# Autodesk Inventor assembly: 200-40-BOGIE-CONNECTOR-REINFORCEMENT-01
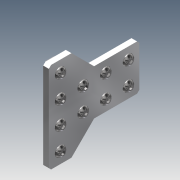
[picture p0: Inventor's stored thumbnail of the model, 180x180]
Saved by Autodesk Inventor 2018.2 (Build 222227000, 227)
## iProperties
Manager: feesmrt
Company: FRANCOR
Part Number: 200-40-BOGIE-CONNECTOR-REINFORCEMENT-01
Project: Rescue Robot
Cost Center: -
Material: Generisch
Document SubType Name: Assembly
Designer: feesmrt
Engineer: feesmrt
Authority: feesmrt
Description: Bogie Connector Verstärkung
Stock Number: 200-40-BOGIE-CONNECTOR-REINFORCEMENT-01
Subject: Rescue Robot
Author: feesmrt
Revision Number: 1
Title: Bogie Connector Verstärkung
## Documents named in this file (4)
- D:\Programmierung\FRANC0R\CAD\02-Rocker-Bogie-Robot\200-ROCKER-BOGIE\200-40-BOGIE-CONNECTOR\200-40-BOGIE-CONNECTOR-REINFORCEMENT-01.iam
- D:\Programmierung\FRANC0R\CAD\02-Rocker-Bogie-Robot\200-ROCKER-BOGIE\200-40-BOGIE-CONNECTOR\200-40-BOGIE-CONNECTOR-06.ipt
- D:\Programmierung\FRANC0R\CAD\02-Rocker-Bogie-Robot\900-COMPONENTS\900-50-PROFILES\900-50-PROFILES-CONN-N6xM5.ipt
- D:\Programmierung\FRANC0R\CAD\02-Rocker-Bogie-Robot\900-COMPONENTS\900-40-SCREWS\900-40-SCREWS-ISO7830_M5x10.ipt
## Components (21 placed, 3 different names)
1. 200-40-BOGIE-CONNECTOR-06:1 — Passend:1, Passend:2, Passend:3, Passend:4, Passend:5, Passend:6, Passend:7, Passend:8, Passend:9, Passend:10, Passend:11, Passend:12, Passend:13, Passend:14, Passend:15, Passend:16, Winkel:1, Winkel:2, Winkel:3, Winkel:4, Winkel:5, Winkel:6, Winkel:7, Winkel:8, Passend:25, Passend:26, Passend:27, Passend:28, Passend:29, Passend:30, Passend:31, Passend:32, Passend:33, Passend:34, Passend:35, Passend:36, Winkel:9, Winkel:10, Passend:39, Passend:40
2. 900-50-PROFILES-CONN-N6xM5:1 — Passend:1, Passend:9, Winkel:4, Passend:24
3. 900-50-PROFILES-CONN-N6xM5:2 — Passend:2, Passend:10, Winkel:3, Passend:23
4. 900-50-PROFILES-CONN-N6xM5:3 — Passend:3, Passend:11, Winkel:2, Passend:22
5. 900-50-PROFILES-CONN-N6xM5:4 — Passend:4, Passend:12, Winkel:1, Passend:21
6. 900-50-PROFILES-CONN-N6xM5:5 — Passend:5, Passend:13, Winkel:5, Passend:19
7. 900-50-PROFILES-CONN-N6xM5:6 — Passend:6, Passend:14, Winkel:7, Passend:20
8. 900-50-PROFILES-CONN-N6xM5:7 — Passend:7, Passend:16, Winkel:6, Passend:18
9. 900-50-PROFILES-CONN-N6xM5:8 — Passend:8, Passend:15, Winkel:8, Passend:17
10. 900-40-SCREWS-ISO7830_M5x10:1 — Passend:17, Passend:25
11. 900-40-SCREWS-ISO7830_M5x10:2 — Passend:18, Passend:26
12. 900-40-SCREWS-ISO7830_M5x10:3 — Passend:20, Passend:27
13. 900-40-SCREWS-ISO7830_M5x10:4 — Passend:19, Passend:28
14. 900-40-SCREWS-ISO7830_M5x10:5 — Passend:21, Passend:29
15. 900-40-SCREWS-ISO7830_M5x10:6 — Passend:22, Passend:30
16. 900-40-SCREWS-ISO7830_M5x10:7 — Passend:23, Passend:31
17. 900-40-SCREWS-ISO7830_M5x10:8 — Passend:24, Passend:32
18. 900-50-PROFILES-CONN-N6xM5:9 — Passend:33, Passend:35, Winkel:10, Passend:37
19. 900-50-PROFILES-CONN-N6xM5:10 — Passend:34, Passend:36, Winkel:9, Passend:38
20. 900-40-SCREWS-ISO7830_M5x10:9 — Passend:37, Passend:39
21. 900-40-SCREWS-ISO7830_M5x10:10 — Passend:38, Passend:40
## Relationships (50: Mate 40, Angle 10)
- Passend:1 [Mate]: 200-40-BOGIE-CONNECTOR-06:1 ↔ 900-50-PROFILES-CONN-N6xM5:1
- Passend:2 [Mate]: 200-40-BOGIE-CONNECTOR-06:1 ↔ 900-50-PROFILES-CONN-N6xM5:2
- Passend:3 [Mate]: 200-40-BOGIE-CONNECTOR-06:1 ↔ 900-50-PROFILES-CONN-N6xM5:3
- Passend:4 [Mate]: 200-40-BOGIE-CONNECTOR-06:1 ↔ 900-50-PROFILES-CONN-N6xM5:4
- Passend:5 [Mate]: 200-40-BOGIE-CONNECTOR-06:1 ↔ 900-50-PROFILES-CONN-N6xM5:5
- Passend:6 [Mate]: 200-40-BOGIE-CONNECTOR-06:1 ↔ 900-50-PROFILES-CONN-N6xM5:6
- Passend:7 [Mate]: 200-40-BOGIE-CONNECTOR-06:1 ↔ 900-50-PROFILES-CONN-N6xM5:7
- Passend:8 [Mate]: 200-40-BOGIE-CONNECTOR-06:1 ↔ 900-50-PROFILES-CONN-N6xM5:8
- Passend:9 [Mate] (1.5 mm): 200-40-BOGIE-CONNECTOR-06:1 ↔ 900-50-PROFILES-CONN-N6xM5:1
- Passend:10 [Mate] (1.5 mm): 200-40-BOGIE-CONNECTOR-06:1 ↔ 900-50-PROFILES-CONN-N6xM5:2
- Passend:11 [Mate] (1.5 mm): 200-40-BOGIE-CONNECTOR-06:1 ↔ 900-50-PROFILES-CONN-N6xM5:3
- Passend:12 [Mate] (1.5 mm): 200-40-BOGIE-CONNECTOR-06:1 ↔ 900-50-PROFILES-CONN-N6xM5:4
- Passend:13 [Mate] (1.5 mm): 200-40-BOGIE-CONNECTOR-06:1 ↔ 900-50-PROFILES-CONN-N6xM5:5
- Passend:14 [Mate] (1.5 mm): 200-40-BOGIE-CONNECTOR-06:1 ↔ 900-50-PROFILES-CONN-N6xM5:6
- Passend:15 [Mate] (1.5 mm): 200-40-BOGIE-CONNECTOR-06:1 ↔ 900-50-PROFILES-CONN-N6xM5:8
- Passend:16 [Mate] (1.5 mm): 200-40-BOGIE-CONNECTOR-06:1 ↔ 900-50-PROFILES-CONN-N6xM5:7
- Winkel:1 [Angle] (0 deg): 200-40-BOGIE-CONNECTOR-06:1 ↔ 900-50-PROFILES-CONN-N6xM5:4
- Winkel:2 [Angle] (0 deg): 200-40-BOGIE-CONNECTOR-06:1 ↔ 900-50-PROFILES-CONN-N6xM5:3
- Winkel:3 [Angle] (0 deg): 200-40-BOGIE-CONNECTOR-06:1 ↔ 900-50-PROFILES-CONN-N6xM5:2
- Winkel:4 [Angle] (0 deg): 200-40-BOGIE-CONNECTOR-06:1 ↔ 900-50-PROFILES-CONN-N6xM5:1
- Winkel:5 [Angle] (0 deg): 200-40-BOGIE-CONNECTOR-06:1 ↔ 900-50-PROFILES-CONN-N6xM5:5
- Winkel:6 [Angle] (0 deg): 200-40-BOGIE-CONNECTOR-06:1 ↔ 900-50-PROFILES-CONN-N6xM5:7
- Winkel:7 [Angle] (0 deg): 200-40-BOGIE-CONNECTOR-06:1 ↔ 900-50-PROFILES-CONN-N6xM5:6
- Winkel:8 [Angle] (0 deg): 200-40-BOGIE-CONNECTOR-06:1 ↔ 900-50-PROFILES-CONN-N6xM5:8
- Passend:17 [Mate]: 900-50-PROFILES-CONN-N6xM5:8 ↔ 900-40-SCREWS-ISO7830_M5x10:1
- Passend:18 [Mate]: 900-50-PROFILES-CONN-N6xM5:7 ↔ 900-40-SCREWS-ISO7830_M5x10:2
- Passend:19 [Mate]: 900-50-PROFILES-CONN-N6xM5:5 ↔ 900-40-SCREWS-ISO7830_M5x10:4
- Passend:20 [Mate]: 900-50-PROFILES-CONN-N6xM5:6 ↔ 900-40-SCREWS-ISO7830_M5x10:3
- Passend:21 [Mate]: 900-50-PROFILES-CONN-N6xM5:4 ↔ 900-40-SCREWS-ISO7830_M5x10:5
- Passend:22 [Mate]: 900-50-PROFILES-CONN-N6xM5:3 ↔ 900-40-SCREWS-ISO7830_M5x10:6
- Passend:23 [Mate]: 900-50-PROFILES-CONN-N6xM5:2 ↔ 900-40-SCREWS-ISO7830_M5x10:7
- Passend:24 [Mate]: 900-50-PROFILES-CONN-N6xM5:1 ↔ 900-40-SCREWS-ISO7830_M5x10:8
- Passend:25 [Mate]: 200-40-BOGIE-CONNECTOR-06:1 ↔ 900-40-SCREWS-ISO7830_M5x10:1
- Passend:26 [Mate]: 200-40-BOGIE-CONNECTOR-06:1 ↔ 900-40-SCREWS-ISO7830_M5x10:2
- Passend:27 [Mate]: 200-40-BOGIE-CONNECTOR-06:1 ↔ 900-40-SCREWS-ISO7830_M5x10:3
- Passend:28 [Mate]: 200-40-BOGIE-CONNECTOR-06:1 ↔ 900-40-SCREWS-ISO7830_M5x10:4
- Passend:29 [Mate]: 200-40-BOGIE-CONNECTOR-06:1 ↔ 900-40-SCREWS-ISO7830_M5x10:5
- Passend:30 [Mate]: 200-40-BOGIE-CONNECTOR-06:1 ↔ 900-40-SCREWS-ISO7830_M5x10:6
- Passend:31 [Mate]: 200-40-BOGIE-CONNECTOR-06:1 ↔ 900-40-SCREWS-ISO7830_M5x10:7
- Passend:32 [Mate]: 200-40-BOGIE-CONNECTOR-06:1 ↔ 900-40-SCREWS-ISO7830_M5x10:8
- Passend:33 [Mate]: 200-40-BOGIE-CONNECTOR-06:1 ↔ 900-50-PROFILES-CONN-N6xM5:9
- Passend:34 [Mate]: 200-40-BOGIE-CONNECTOR-06:1 ↔ 900-50-PROFILES-CONN-N6xM5:10
- Passend:35 [Mate] (1.5 mm): 200-40-BOGIE-CONNECTOR-06:1 ↔ 900-50-PROFILES-CONN-N6xM5:9
- Passend:36 [Mate] (1.5 mm): 200-40-BOGIE-CONNECTOR-06:1 ↔ 900-50-PROFILES-CONN-N6xM5:10
- Winkel:9 [Angle] (0 deg): 200-40-BOGIE-CONNECTOR-06:1 ↔ 900-50-PROFILES-CONN-N6xM5:10
- Winkel:10 [Angle] (0 deg): 200-40-BOGIE-CONNECTOR-06:1 ↔ 900-50-PROFILES-CONN-N6xM5:9
- Passend:37 [Mate]: 900-50-PROFILES-CONN-N6xM5:9 ↔ 900-40-SCREWS-ISO7830_M5x10:9
- Passend:38 [Mate]: 900-50-PROFILES-CONN-N6xM5:10 ↔ 900-40-SCREWS-ISO7830_M5x10:10
- Passend:39 [Mate]: 200-40-BOGIE-CONNECTOR-06:1 ↔ 900-40-SCREWS-ISO7830_M5x10:9
- Passend:40 [Mate]: 200-40-BOGIE-CONNECTOR-06:1 ↔ 900-40-SCREWS-ISO7830_M5x10:10
